# Autodesk Inventor assembly: JLNSK50
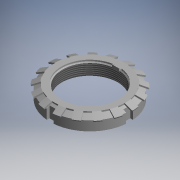
[picture p0: Inventor's stored thumbnail of the model, 180x180]
Saved by Autodesk Inventor 2017.3 (Build 213256000, 256)
## iProperties
Category: PARTsolutions
Company: MISUMI
Part Number: JLNSK50
Catalog Web Link: www.cadenas.de
Description: JLNK, JLNSK-Nuts for Bearings - Stainless Steel /E/ Tooth Lock Washer Set
Vendor: MISUMI
Document SubType Name: Assembly
Designer: partserver
Manufacturer: MISUMI
Mass: 22.263 g
Surface Area: 116.953 cm^2
Volume: 22.263 cm^3
Density: 1 g/cm^3
Title: JLNSK50
Author: Cadenas PARTsolutions
Comments: Nuts for Bearings - Stainless Steel /E/ Tooth Lock Washer Set
PSOL_IDENT_0: {$CADENAS_DATA\23d-libs\misumi\metric\12_bearing_holders\jlnsk_asmtab.prj},169 {VTYP=3D},{STYP=ASSTA
PSOL_IDENT_1: B},{NB=JLNSK50},{LINA=JLNSK50},{NN=JLNK, JLNSK},{DATE=30.10.2020 16:03:41},{GEOMDATE=06.07.2009},{VE
PSOL_IDENT_2: RSION=},{LINEID=110},{WBVAR=MATN},{WBNUMERIC=}  {NB=JLNSK50},{LINA=JLNSK50},{KT=DUMMY},{PN=JLNSK50},
PSOL_IDENT_3: {NO=50},{TS=2},{TYPE=JLNSK},{MATN=SUS304},{MATNALG='1018','1018 Carbon Steel','SUS304','304 Stainles
PSOL_IDENT_4: s Steel'},{MATW=304 Stainless Steel},{M=50 x 1.5},{M1=50},{PITCH=1.500},{D1=70},{D2=61},{B=11},{DD=6
PSOL_IDENT_5: 5},{S=6},{T=2.5},{RWS=161.5},{RWN=0.0},{PPATH=jlnk_asmtpl.prj},{DD1=50},{KK=47.5},{S1=6},{S2=6},{TT=
PSOL_IDENT_6: 1.2},{V=2.5},{D3=74},{D4=61},{NOTH=17}
NB: JLNSK50
NN: JLNK, JLNSK
NT: Nuts for Bearings - Stainless Steel /E/ Tooth Lock Washer Set
NBSYN: $PN.
LINA: JLNSK50
CATALOG: Misumi
PN: JLNSK50
NO: 50
MATN: 304 Stainless Steel
MATW: 304 Stainless Steel
M: 50 x 1.5
D1: 70
D2: 61
B: 11
DD: 65
S: 6
T: 2.5
RWS: 161.5
RWN: 0
DD1: 50
KK: 47.5
S1: 6
S2: 6
TT: 1.2
V: 2.5
D3: 74
D4: 61
NOTH: 17
SUPPLIER: MISUMI
ARTICLENO: JLNSK50
BOMINFO: JLNSK50
CREATOR: CADENAS GmbH
## Documents named in this file (3)
- e:\temp\worker_19\temp\exporttempdir_264_36_dlq8i\format_0\JLNSK50.iam
- e:\temp\worker_19\temp\exporttempdir_264_36_dlq8i\format_0\JLNSK50nut.ipt
- e:\temp\worker_19\temp\exporttempdir_264_36_dlq8i\format_0\Washer50w.ipt
## Components (2 placed, 2 different names)
1. JLNSK50nut:1 — wash_to_nut_XY@1 <-> washer_XY@2, wash_to_nut_Z@1 <-> washer_Z@2, wash_to_nut_YZ@1 <-> washer_YZ@2
2. Washer50w:1 — wash_to_nut_XY@1 <-> washer_XY@2, wash_to_nut_Z@1 <-> washer_Z@2, wash_to_nut_YZ@1 <-> washer_YZ@2
## Relationships (3: Flush 1, Mate 1, Angle 1)
- wash_to_nut_XY@1 <-> washer_XY@2 [Flush]: JLNSK50nut:1 ↔ Washer50w:1
- wash_to_nut_Z@1 <-> washer_Z@2 [Mate]: JLNSK50nut:1 ↔ Washer50w:1
- wash_to_nut_YZ@1 <-> washer_YZ@2 [Angle] (0 deg): JLNSK50nut:1 ↔ Washer50w:1
